# Autodesk Inventor assembly: Assembly2
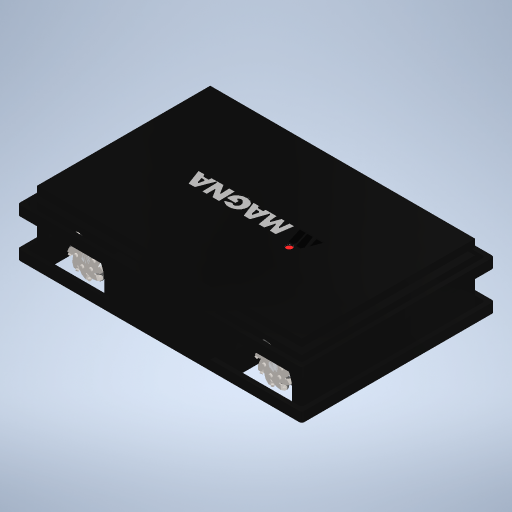
[picture p0: Inventor's stored thumbnail of the model, 512x512]
Saved by Autodesk Inventor 2024 (Build 280153000, 153)
## iProperties
Created: 2024-04-03
Part Number: Assembly2
Document SubType Name: Assembly
Designer: Gabek
Author: Gabek
## Documents named in this file (3)
- D:\factory-digital-twin\src\assets\glb_models\Assembly2.iam
- D:\factory-digital-twin\src\assets\glb_models\platform.ipt
- D:\factory-digital-twin\src\assets\glb_models\wheel.ipt
## Components (5 placed, 2 different names)
1. platform:1 — Mate:1, Mate:2, Mate:3, Mate:4, Mate:5, Mate:6, Mate:7, Mate:8, Mate:9, Mate:10, Mate:11
2. wheel:1 — Mate:2, Mate:5
3. wheel:2 — Mate:3, Mate:4
4. wheel:3 — Mate:1, Mate:6
5. wheel:4 — Mate:7, Mate:8
## Relationships (11: Mate 11)
- Mate:1: platform:1 ↔ wheel:3
- Mate:2: platform:1 ↔ wheel:1
- Mate:3: platform:1 ↔ wheel:2
- Mate:4: platform:1 ↔ wheel:2
- Mate:5: platform:1 ↔ wheel:1
- Mate:6: platform:1 ↔ wheel:3
- Mate:7: platform:1 ↔ wheel:4
- Mate:8: platform:1 ↔ wheel:4
- Mate:9 (12.7 mm): platform:1
- Mate:10: platform:1
- Mate:11: platform:1
